# Autodesk Inventor assembly: 20X20 carege assembly
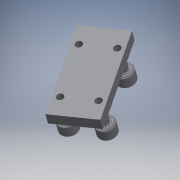
[picture p0: Inventor's stored thumbnail of the model, 180x180]
Saved by Autodesk Inventor 2019 (Build 230136000, 136)
## iProperties
Created: 2018-12-06
Part Number: 20X20 carege assembly
Document SubType Name: Assembly
Designer: User
Author: User
## Documents named in this file (4)
- C:\Robotics\CAD\2018-19_CAD\Collection\20X20 carege assembly.iam
- C:\Robotics\CAD\2018-19_CAD\Collection\20X20 carege.ipt
- C:\Robotics\CAD\COTSParts\Actobotics\615 parts\615454 assembly.ipt
- C:\Robotics\CAD\COTSParts\Actobotics\633 parts\633177.ipt
## Components (9 placed, 3 different names)
1. 20X20 carege:1 — Mate:1, Mate:2, Mate:3, Mate:4, Mate:5, Mate:6, Mate:7, Mate:8
2. 615454 assembly:3 — Insert:4
3. 615454 assembly:5 — Insert:3
4. 615454 assembly:6 — Insert:2
5. 615454 assembly:7 — Insert:1
6. 633177:1 — Mate:3, Mate:8, Insert:2
7. 633177:2 — Mate:1, Mate:2, Insert:1
8. 633177:3 — Mate:5, Mate:6, Insert:4
9. 633177:4 — Mate:4, Mate:7, Insert:3
## Relationships (12: Mate 8, Insert 4)
- Mate:1: 20X20 carege:1 ↔ 633177:2
- Mate:2: 20X20 carege:1 ↔ 633177:2
- Mate:3: 20X20 carege:1 ↔ 633177:1
- Mate:4: 20X20 carege:1 ↔ 633177:4
- Mate:5: 20X20 carege:1 ↔ 633177:3
- Mate:6: 20X20 carege:1 ↔ 633177:3
- Mate:7: 20X20 carege:1 ↔ 633177:4
- Mate:8: 20X20 carege:1 ↔ 633177:1
- Insert:1: 615454 assembly:7 ↔ 633177:2
- Insert:2: 615454 assembly:6 ↔ 633177:1
- Insert:3: 615454 assembly:5 ↔ 633177:4
- Insert:4: 615454 assembly:3 ↔ 633177:3
